# Autodesk Inventor assembly: assem_finger_thumb_linact_v2
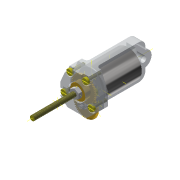
[picture p0: Inventor's stored thumbnail of the model, 180x180]
Saved by Autodesk Inventor 2014 (Build 180170000, 170)
## iProperties
Created: 2015-05-22
Part Number: assem_finger_thumb_linact_v2
Document SubType Name: Assembly
Designer: Martin
Author: Martin
## Documents named in this file (11)
- C:\Users\Martin\Dropbox\biohand-mec\biohand_v1\fingers\thumb\assem_finger_thumb_linact_v2.iam
- C:\Users\Martin\Dropbox\biohand-mec\biohand_v1\fingers\thumb\linact_thumb_cage.ipt
- C:\Users\Martin\Dropbox\biohand-mec\biohand_v1\misc\motor_servo.ipt
- C:\Users\Martin\Dropbox\biohand-mec\biohand_v1\misc\servo_gear_1.ipt
- C:\Users\Martin\Dropbox\biohand-mec\biohand_v1\fingers\thumb\linact_thumb_front.ipt
- C:\Users\Martin\Dropbox\biohand-mec\biohand_v1\misc\servo_gear_2.ipt
- C:\Users\Martin\Dropbox\biohand-mec\biohand_v1\misc\m3_30_screw.ipt
- C:\Users\Martin\Dropbox\biohand-mec\biohand_v1\misc\m2_8_screw.ipt
- C:\Users\Martin\Dropbox\biohand-mec\biohand_v1\misc\m3_nut.ipt
- C:\Users\Martin\Dropbox\biohand-mec\biohand_v1\misc\m2_4_screw.ipt
- C:\Users\Martin\Dropbox\biohand-mec\biohand_v1\misc\servo_small_dowel.ipt
## Components (14 placed, 10 different names)
1. linact_thumb_cage:1 — Insert:1, Mate:1, Flush:1, Insert:2, Insert:10, Insert:11
2. motor_servo:1 — Insert:1, Mate:1
3. servo_gear_1:1 — Insert:2
4. servo_gear_2:1 — Insert:3, Insert:4, Insert:9
5. linact_thumb_front:1 — Flush:2, Flush:3, Insert:4, Insert:5, Insert:6, Insert:7, Insert:8, Insert:12
6. m3_30_screw:1 — Insert:3
7. m2_8_screw:1 — Insert:5
8. m2_8_screw:2 — Insert:6
9. m2_8_screw:3 — Insert:8
10. m2_8_screw:4 — Insert:7
11. m3_nut:1 — Insert:9
12. m2_4_screw:1 — Insert:10
13. m2_4_screw:2 — Insert:11
14. servo_small_dowel:1 — Insert:12
## Relationships (16: Insert 12, Flush 3, Mate 1)
- Insert:1: linact_thumb_cage:1 ↔ motor_servo:1
- Mate:1: linact_thumb_cage:1 ↔ motor_servo:1
- Flush:1 (2.8 mm): linact_thumb_cage:1
- Insert:2 (0.5 mm): linact_thumb_cage:1 ↔ servo_gear_1:1
- Flush:2: linact_thumb_front:1
- Flush:3: linact_thumb_front:1
- Insert:3: servo_gear_2:1 ↔ m3_30_screw:1
- Insert:4: servo_gear_2:1 ↔ linact_thumb_front:1
- Insert:5: linact_thumb_front:1 ↔ m2_8_screw:1
- Insert:6: linact_thumb_front:1 ↔ m2_8_screw:2
- Insert:7: linact_thumb_front:1 ↔ m2_8_screw:4
- Insert:8: linact_thumb_front:1 ↔ m2_8_screw:3
- Insert:9: servo_gear_2:1 ↔ m3_nut:1
- Insert:10: linact_thumb_cage:1 ↔ m2_4_screw:1
- Insert:11: linact_thumb_cage:1 ↔ m2_4_screw:2
- Insert:12 (-0.75 mm): linact_thumb_front:1 ↔ servo_small_dowel:1
